# Autodesk Inventor assembly: Matchboxscope_VCM_v1
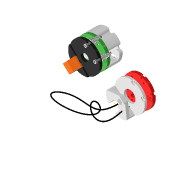
[picture p0: Inventor's stored thumbnail of the model, 180x180]
Saved by Autodesk Inventor 2022 (Build 260153000, 153)
## iProperties
Created: 2022-04-02
Part Number: Matchboxscope_VCM_v1
Document SubType Name: Assembly
Designer: Prakash Lab
Author: Prakash Lab
## Documents named in this file (13)
- C:\Users\diederichbenedict\Dropbox\Dokumente\Promotion\PROJECTS\Matchboxscope\INVENTOR\MATCHBOXSCOPE\Matchboxscope_VCM_v1.iam
- C:\Users\diederichbenedict\Dropbox\Dokumente\Promotion\PROJECTS\Matchboxscope\INVENTOR\MATCHBOXSCOPE\Matchboxscope_Lightperiscope_V0.ipt
- C:\Users\diederichbenedict\Dropbox\Dokumente\Promotion\PROJECTS\Matchboxscope\INVENTOR\MATCHBOXSCOPE\Matchboxscope_bottom_v0.ipt
- C:\Users\diederichbenedict\Dropbox\Dokumente\Promotion\PROJECTS\Matchboxscope\INVENTOR\MATCHBOXSCOPE\00_ESP3-CAM.iam
- C:\Users\diederichbenedict\Dropbox\Dokumente\Promotion\PROJECTS\Matchboxscope\INVENTOR\MATCHBOXSCOPE\00_Powerbank.ipt
- C:\Users\diederichbenedict\Dropbox\Dokumente\Promotion\PROJECTS\Matchboxscope\INVENTOR\MATCHBOXSCOPE\00_spring.ipt
- C:\Users\diederichbenedict\Documents\Inventor\Content Center Files\R2022\de-DE\DIN 912\DIN 912 - M3 x 0.5 x 25 x 18.ipt
- C:\Users\diederichbenedict\Dropbox\Dokumente\Promotion\PROJECTS\Matchboxscope\INVENTOR\MATCHBOXSCOPE\Matchboxscope_sample_universal.ipt
- C:\Users\diederichbenedict\Dropbox\Dokumente\Promotion\PROJECTS\Matchboxscope\INVENTOR\MATCHBOXSCOPE\Matchboxscope_middle2_m12VCMLens_v2.ipt
- C:\Users\diederichbenedict\Dropbox\Dokumente\Promotion\PROJECTS\Matchboxscope\INVENTOR\MATCHBOXSCOPE\Matchboxscope_middle2_v2.ipt
- C:\Users\diederichbenedict\Dropbox\Dokumente\Promotion\PROJECTS\Matchboxscope\INVENTOR\MATCHBOXSCOPE\Anglerfish_Cameraspacer.ipt
- C:\Users\diederichbenedict\Dropbox\Dokumente\Promotion\PROJECTS\Matchboxscope\INVENTOR\MATCHBOXSCOPE\Matchboxscope_sample_universal_toslink.ipt
- C:\Users\diederichbenedict\Dropbox\Dokumente\Promotion\PROJECTS\Matchboxscope\INVENTOR\MATCHBOXSCOPE\00_Toslink.ipt
## Components (20 placed, 12 different names)
1. Matchboxscope_Lightperiscope_V0:1 — Einfügen:19
2. Matchboxscope_bottom_v0:1 — Mate:1, Mate:2, Mate:3, Mate:4, Flush:1, Einfügen:11, Passend:7, Winkel:3
3. 00_ESP3-CAM:1 [sub-assembly] — Mate:4, Flush:1
4. Matchboxscope_sample_universal:2 — Winkel:3, Einfügen:12, Einfügen:13, Einfügen:14, Einfügen:15, Einfügen:16, Einfügen:17, Einfügen:19
5. 00_Powerbank:1
6. 00_spring:1 — Einfügen:17
7. DIN 912 - ersetzt durch DIN EN ISO 4762 M3 x 25:1 — Einfügen:14
8. DIN 912 - ersetzt durch DIN EN ISO 4762 M3 x 25:2 — Einfügen:12
9. DIN 912 - ersetzt durch DIN EN ISO 4762 M3 x 25:3 — Einfügen:13
10. 00_spring:3 — Einfügen:15
11. 00_spring:4 — Einfügen:16
12. DIN 912 - ersetzt durch DIN EN ISO 4762 M3 x 25:4
13. DIN 912 - ersetzt durch DIN EN ISO 4762 M3 x 25:5
14. DIN 912 - ersetzt durch DIN EN ISO 4762 M3 x 25:6
15. DIN 912 - ersetzt durch DIN EN ISO 4762 M3 x 25:7
16. Matchboxscope_middle2_m12VCMLens_v2:1 — Einfügen:11, Passend:7
17. Matchboxscope_middle2_v2:1 — Einfügen:18
18. Anglerfish_Cameraspacer:1
19. Matchboxscope_sample_universal_toslink:1 — Einfügen:18, Einfügen:20
20. 00_Toslink:1 — Einfügen:20
## Relationships (17: Insert 10, Mate 5, Flush 1, Angle 1)
- Mate:1: Matchboxscope_bottom_v0:1
- Mate:2: Matchboxscope_bottom_v0:1
- Mate:3: Matchboxscope_bottom_v0:1
- Mate:4: Matchboxscope_bottom_v0:1 ↔ 00_ESP3-CAM:1
- Flush:1: Matchboxscope_bottom_v0:1 ↔ 00_ESP3-CAM:1
- Einfügen:11 [Insert]: Matchboxscope_bottom_v0:1 ↔ Matchboxscope_middle2_m12VCMLens_v2:1
- Passend:7 [Mate]: Matchboxscope_bottom_v0:1 ↔ Matchboxscope_middle2_m12VCMLens_v2:1
- Winkel:3 [Angle] (45 deg): Matchboxscope_bottom_v0:1 ↔ Matchboxscope_sample_universal:2
- Einfügen:12 [Insert]: Matchboxscope_sample_universal:2 ↔ DIN 912 - ersetzt durch DIN EN ISO 4762 M3 x 25:2
- Einfügen:13 [Insert]: Matchboxscope_sample_universal:2 ↔ DIN 912 - ersetzt durch DIN EN ISO 4762 M3 x 25:3
- Einfügen:14 [Insert]: Matchboxscope_sample_universal:2 ↔ DIN 912 - ersetzt durch DIN EN ISO 4762 M3 x 25:1
- Einfügen:15 [Insert]: Matchboxscope_sample_universal:2 ↔ 00_spring:3
- Einfügen:16 [Insert]: Matchboxscope_sample_universal:2 ↔ 00_spring:4
- Einfügen:17 [Insert]: Matchboxscope_sample_universal:2 ↔ 00_spring:1
- Einfügen:18 [Insert] (10 mm): Matchboxscope_middle2_v2:1 ↔ Matchboxscope_sample_universal_toslink:1
- Einfügen:19 [Insert]: Matchboxscope_Lightperiscope_V0:1 ↔ Matchboxscope_sample_universal:2
- Einfügen:20 [Insert]: Matchboxscope_sample_universal_toslink:1 ↔ 00_Toslink:1
